# Autodesk Inventor assembly: ASY Рама под жмых
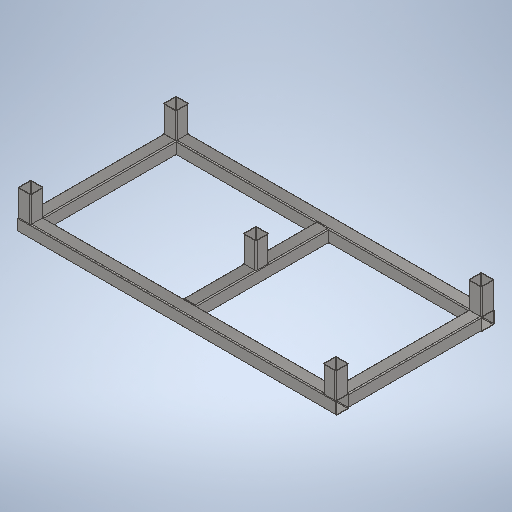
[picture p0: Inventor's stored thumbnail of the model, 512x512]
Saved by Autodesk Inventor 2025 (Build 290162010, 162A)
## iProperties
Created: 2025-02-02
Part Number: ASY Рама под жмых
Document SubType Name: Assembly
Designer: pokla
Author: pokla
## Documents named in this file (3)
- C:\Users\pokla\Documents\Inventor\Отстойник осветлитель\Manturovo_Se-clar-Gleb\ASY Рама под жмых.iam
- C:\Users\pokla\Documents\Inventor\Отстойник осветлитель\Manturovo_Se-clar-Gleb\ASY Рама под жмых верх.iam
- C:\Users\pokla\Documents\Inventor\Отстойник осветлитель\Manturovo_Se-clar-Gleb\ISO 4019 - 50x50x2 - 100.ipt
## Components (6 placed, 2 different names)
1. ASY Рама под жмых верх:1 [sub-assembly] — Rigid:1, Rigid:2
2. ISO 4019 - 50x50x2 - 100:2 — Rigid:1
3. ISO 4019 - 50x50x2 - 100:1 — Rigid:2
4. ISO 4019 - 50x50x2 - 100:3
5. ISO 4019 - 50x50x2 - 100:4
6. ISO 4019 - 50x50x2 - 100:5
## Component patterns: (4 elements, first: ISO 4019 - 50x50x2 - 100:1)
## Relationships (2: WeldJoint 2)
- Rigid:1 [WeldJoint]: ASY Рама под жмых верх:1 ↔ ISO 4019 - 50x50x2 - 100:2
- Rigid:2 [WeldJoint]: ASY Рама под жмых верх:1 ↔ ISO 4019 - 50x50x2 - 100:1
